# Autodesk Inventor assembly: Robot Réduit
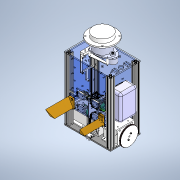
[picture p0: Inventor's stored thumbnail of the model, 180x180]
Saved by Autodesk Inventor 2022 (Build 260153000, 153)
## iProperties
Created: 2022-04-26
Part Number: Robot Réduit
Document SubType Name: Assembly
Designer: victo
Author: victo
## Documents named in this file (25)
- C:\Users\victo\Desktop\Documents\ENSTA\Cours ENSTA\2A\PIE\Modélisation\Robot réduit\Robot Réduit.iam
- C:\Users\victo\Desktop\Documents\ENSTA\Cours ENSTA\2A\PIE\Modélisation\Robot réduit\Base robot réduit.ipt
- C:\Users\victo\Desktop\Documents\ENSTA\Cours ENSTA\2A\PIE\Modélisation\Robot réduit\Biellette moteur-doigts.ipt
- C:\Users\victo\Desktop\Documents\ENSTA\Cours ENSTA\2A\PIE\Modélisation\Robot réduit\Support AX 12A.ipt
- C:\Users\victo\Desktop\Documents\ENSTA\Cours ENSTA\2A\PIE\Modélisation\Propre 0 - Base roue batteries\Moteur déplacement gauche.iam
- C:\Users\victo\Desktop\Documents\ENSTA\Cours ENSTA\2A\PIE\Modélisation\Propre 0 - Base roue batteries\Moteur déplacement droit.iam
- C:\Users\victo\Desktop\Documents\ENSTA\Cours ENSTA\2A\PIE\Modélisation\Robot réduit\Support AX 12A haut.ipt
- C:\Users\victo\Desktop\Documents\ENSTA\Cours ENSTA\2A\PIE\Modélisation\Robot réduit\Batterie et Support Vertical Réduit.iam
- C:\Users\victo\Desktop\Documents\ENSTA\Cours ENSTA\2A\PIE\Modélisation\Robot réduit\Profilés du réduit 20x20.ipt
- C:\Users\victo\Desktop\Documents\ENSTA\Cours ENSTA\2A\PIE\Modélisation\Robot réduit\Support rotation.ipt
- C:\Users\victo\Desktop\Documents\ENSTA\Cours ENSTA\2A\PIE\Modélisation\Robot réduit\Plaque trans.ipt
- C:\Users\victo\Desktop\Documents\ENSTA\Cours ENSTA\2A\PIE\Modélisation\Robot réduit\Doigt droit.ipt
- C:\Users\victo\Desktop\Documents\ENSTA\Cours ENSTA\2A\PIE\Modélisation\Pieces commerce\AX 12AAX-12A_[Servo.ipt
- C:\Users\victo\Desktop\Documents\ENSTA\Cours ENSTA\2A\PIE\Modélisation\Robot réduit\Biellette support-doigts.ipt
- C:\Users\victo\Desktop\Documents\ENSTA\Cours ENSTA\2A\PIE\Modélisation\Robot réduit\Doigt gauche.ipt
- C:\Users\victo\Desktop\Documents\ENSTA\Cours ENSTA\2A\PIE\Modélisation\Robot réduit\Support Vis rotation.ipt
- C:\Users\victo\Desktop\Documents\ENSTA\Cours ENSTA\2A\PIE\Modélisation\Robot réduit\ASS_Roue_Libre-20220506T114758Z-001\ASS_Roue_Libre\ASS_Roue_Libre.iam
- C:\Users\victo\Desktop\Documents\ENSTA\Cours ENSTA\2A\PIE\Modélisation\Robot réduit\Etage robot réduit.ipt
- C:\Users\victo\Desktop\Documents\ENSTA\Cours ENSTA\2A\PIE\Modélisation\Robot réduit\Support_LIDAR.ipt
- C:\Users\victo\Desktop\Documents\ENSTA\Cours ENSTA\2A\PIE\Modélisation\Robot réduit\Support_Raspberry.ipt
- C:\Users\victo\Desktop\Documents\ENSTA\Cours ENSTA\2A\PIE\Modélisation\Robot réduit\Chapeau Haut.stl.ipt
- C:\Users\victo\Desktop\Documents\ENSTA\Cours ENSTA\2A\PIE\Modélisation\Robot réduit\rplidar_main.ipt
- C:\Users\victo\Desktop\Documents\ENSTA\Cours ENSTA\2A\PIE\Modélisation\Robot réduit\Plaques latétales\Plaque avant.ipt
- C:\Users\victo\Desktop\Documents\ENSTA\Cours ENSTA\2A\PIE\Modélisation\Robot réduit\Plaques latétales\Plaque arrière.ipt
- C:\Users\victo\Desktop\Documents\ENSTA\Cours ENSTA\2A\PIE\Modélisation\Robot réduit\Plaques latétales\Plaque gauche.ipt
## Components (35 placed, 24 different names)
1. Base robot réduit:1 — Logement:3, Placage:2, Logement:4, Placage:3, Logement:6, Placage:5, Logement:9, Logement:10, Logement:11, Logement:12, Angle:1, Angle:2, Angle:3, Angle:4, Placage:24, Affleurement:1, Placage:25, Affleurement:2
2. Moteur déplacement droit:1 [sub-assembly] — Logement:4, Placage:3
3. Moteur déplacement gauche:1 [sub-assembly] — Logement:3, Placage:2, Logement:7, Placage:6
4. Support AX 12A:1 — Logement:2, Logement:5, Placage:4, Logement:19, Placage:14, Placage:15, Logement:24, Placage:22
5. Support AX 12A haut:1 — Logement:5, Placage:4, Logement:6, Placage:5, Logement:8, Logement:20, Placage:13, Placage:16, Placage:23, Logement:25
6. Biellette moteur-doigts:1 — Logement:2, Logement:17, Placage:19, Placage:20
7. Batterie et Support Vertical Réduit:1 [sub-assembly] — Logement:7, Placage:6
8. Biellette moteur-doigts:2 — Logement:8, Placage:11, Placage:17, Placage:18
9. Profilés du réduit 20x20:1 — Logement:12, Angle:4
10. Profilés du réduit 20x20:2 — Logement:9, Angle:1, Logement:26
11. Profilés du réduit 20x20:3 — Logement:10, Angle:3, Placage:26
12. Profilés du réduit 20x20:4 — Logement:11, Angle:2
13. Support rotation:1 — Logement:14, Placage:9, Logement:17
14. Support rotation:2 — Logement:13, Placage:10, Logement:22
15. Plaque trans:1 — Logement:13, Logement:14, Logement:15, Logement:16, Placage:7, Placage:8, Placage:9, Placage:10, Logement:18, Placage:12, Logement:23, Placage:21
16. Support rotation:3 — Logement:15, Placage:8, Logement:21
17. Support rotation:4 — Logement:16, Placage:7, Placage:11
18. Doigt droit:1 — Logement:18, Placage:12
19. AX 12AAX-12A_[Servo:1 — Logement:19, Placage:14, Placage:19, Placage:20
20. AX 12AAX-12A_[Servo:2 — Logement:20, Placage:13, Placage:17, Placage:18
21. Biellette support-doigts:1 — Logement:21, Placage:15
22. Biellette support-doigts:2 — Logement:22, Placage:16
23. Doigt gauche:1 — Logement:23, Placage:21
24. Support Vis rotation:1 — Logement:24, Placage:22
25. Support Vis rotation:2 — Placage:23, Logement:25
26. ASS_Roue_Libre:1 [sub-assembly] — Placage:24, Affleurement:1
27. ASS_Roue_Libre:2 [sub-assembly] — Placage:25, Affleurement:2
28. Etage robot réduit:1 — Logement:26, Placage:26, Placage:27, Placage:28, Placage:29, Logement:27, Placage:30, Placage:31, Placage:32, Placage:33, Placage:35, Affleurement:3, Placage:36, Affleurement:38, Placage:37, Affleurement:39
29. Support_LIDAR:1 — Placage:27, Placage:28, Placage:29, Logement:28, Placage:34
30. Support_Raspberry:1 — Logement:27, Placage:30
31. Chapeau Haut.stl:1 — Placage:31, Placage:32, Placage:33
32. rplidar_main:1 — Logement:28, Placage:34
33. Plaque avant:1 — Placage:35, Affleurement:3
34. Plaque arrière:1 — Placage:36, Affleurement:38
35. Plaque gauche:1 — Placage:37, Affleurement:39
## Relationships (72: Mate 36, Insert 27, Flush 5, Angle 4)
- Logement:2 [Insert]: Support AX 12A:1 ↔ Biellette moteur-doigts:1
- Logement:3 [Insert]: Base robot réduit:1 ↔ Moteur déplacement gauche:1
- Placage:2 [Mate]: Base robot réduit:1 ↔ Moteur déplacement gauche:1
- Logement:4 [Insert]: Base robot réduit:1 ↔ Moteur déplacement droit:1
- Placage:3 [Mate]: Base robot réduit:1 ↔ Moteur déplacement droit:1
- Logement:5 [Insert]: Support AX 12A:1 ↔ Support AX 12A haut:1
- Placage:4 [Mate]: Support AX 12A:1 ↔ Support AX 12A haut:1
- Logement:6 [Insert]: Base robot réduit:1 ↔ Support AX 12A haut:1
- Placage:5 [Mate]: Base robot réduit:1 ↔ Support AX 12A haut:1
- Logement:7 [Insert]: Moteur déplacement gauche:1 ↔ Batterie et Support Vertical Réduit:1
- Placage:6 [Mate]: Moteur déplacement gauche:1 ↔ Batterie et Support Vertical Réduit:1
- Logement:8 [Insert]: Support AX 12A haut:1 ↔ Biellette moteur-doigts:2
- Logement:9 [Insert]: Base robot réduit:1 ↔ Profilés du réduit 20x20:2
- Logement:10 [Insert]: Base robot réduit:1 ↔ Profilés du réduit 20x20:3
- Logement:11 [Insert]: Base robot réduit:1 ↔ Profilés du réduit 20x20:4
- Logement:12 [Insert]: Base robot réduit:1 ↔ Profilés du réduit 20x20:1
- Angle:1 (0 deg): Base robot réduit:1 ↔ Profilés du réduit 20x20:2
- Angle:2 (0 deg): Base robot réduit:1 ↔ Profilés du réduit 20x20:4
- Angle:3 (0 deg): Base robot réduit:1 ↔ Profilés du réduit 20x20:3
- Angle:4 (0 deg): Base robot réduit:1 ↔ Profilés du réduit 20x20:1
- Logement:13 [Insert]: Support rotation:2 ↔ Plaque trans:1
- Logement:14 [Insert]: Support rotation:1 ↔ Plaque trans:1
- Logement:15 [Insert]: Plaque trans:1 ↔ Support rotation:3
- Logement:16 [Insert]: Plaque trans:1 ↔ Support rotation:4
- Placage:7 [Mate]: Plaque trans:1 ↔ Support rotation:4
- Placage:8 [Mate]: Plaque trans:1 ↔ Support rotation:3
- Placage:9 [Mate]: Support rotation:1 ↔ Plaque trans:1
- Placage:10 [Mate]: Support rotation:2 ↔ Plaque trans:1
- Logement:17 [Insert] (0.5 mm): Biellette moteur-doigts:1 ↔ Support rotation:1
- Placage:11 [Mate]: Biellette moteur-doigts:2 ↔ Support rotation:4
- Logement:18 [Insert]: Plaque trans:1 ↔ Doigt droit:1
- Placage:12 [Mate]: Plaque trans:1 ↔ Doigt droit:1
- Logement:19 [Insert]: Support AX 12A:1 ↔ AX 12AAX-12A_[Servo:1
- Logement:20 [Insert]: Support AX 12A haut:1 ↔ AX 12AAX-12A_[Servo:2
- Placage:13 [Mate]: Support AX 12A haut:1 ↔ AX 12AAX-12A_[Servo:2
- Placage:14 [Mate]: Support AX 12A:1 ↔ AX 12AAX-12A_[Servo:1
- Logement:21 [Insert] (0.5 mm): Support rotation:3 ↔ Biellette support-doigts:1
- Logement:22 [Insert] (0.5 mm): Support rotation:2 ↔ Biellette support-doigts:2
- Placage:15 [Mate]: Support AX 12A:1 ↔ Biellette support-doigts:1
- Placage:16 [Mate]: Support AX 12A haut:1 ↔ Biellette support-doigts:2
- Placage:17 [Mate]: Biellette moteur-doigts:2 ↔ AX 12AAX-12A_[Servo:2
- Placage:18 [Mate]: Biellette moteur-doigts:2 ↔ AX 12AAX-12A_[Servo:2
- Placage:19 [Mate]: Biellette moteur-doigts:1 ↔ AX 12AAX-12A_[Servo:1
- Placage:20 [Mate]: Biellette moteur-doigts:1 ↔ AX 12AAX-12A_[Servo:1
- Logement:23 [Insert]: Plaque trans:1 ↔ Doigt gauche:1
- Placage:21 [Mate]: Plaque trans:1 ↔ Doigt gauche:1
- Logement:24 [Insert]: Support AX 12A:1 ↔ Support Vis rotation:1
- Placage:22 [Mate]: Support AX 12A:1 ↔ Support Vis rotation:1
- Placage:23 [Mate]: Support AX 12A haut:1 ↔ Support Vis rotation:2
- Logement:25 [Insert]: Support AX 12A haut:1 ↔ Support Vis rotation:2
- Placage:24 [Mate]: Base robot réduit:1 ↔ ASS_Roue_Libre:1
- Affleurement:1 [Flush]: Base robot réduit:1 ↔ ASS_Roue_Libre:1
- Placage:25 [Mate]: Base robot réduit:1 ↔ ASS_Roue_Libre:2
- Affleurement:2 [Flush]: Base robot réduit:1 ↔ ASS_Roue_Libre:2
- Logement:26 [Insert]: Profilés du réduit 20x20:2 ↔ Etage robot réduit:1
- Placage:26 [Mate]: Profilés du réduit 20x20:3 ↔ Etage robot réduit:1
- Placage:27 [Mate]: Etage robot réduit:1 ↔ Support_LIDAR:1
- Placage:28 [Mate]: Etage robot réduit:1 ↔ Support_LIDAR:1
- Placage:29 [Mate]: Etage robot réduit:1 ↔ Support_LIDAR:1
- Logement:27 [Insert]: Etage robot réduit:1 ↔ Support_Raspberry:1
- Placage:30 [Mate]: Etage robot réduit:1 ↔ Support_Raspberry:1
- Placage:31 [Mate]: Etage robot réduit:1 ↔ Chapeau Haut.stl:1
- Placage:32 [Mate]: Etage robot réduit:1 ↔ Chapeau Haut.stl:1
- Placage:33 [Mate] (70 mm): Etage robot réduit:1 ↔ Chapeau Haut.stl:1
- Logement:28 [Insert]: Support_LIDAR:1 ↔ rplidar_main:1
- Placage:34 [Mate]: Support_LIDAR:1 ↔ rplidar_main:1
- Placage:35 [Mate]: Etage robot réduit:1 ↔ Plaque avant:1
- Affleurement:3 [Flush]: Etage robot réduit:1 ↔ Plaque avant:1
- Placage:36 [Mate]: Etage robot réduit:1 ↔ Plaque arrière:1
- Affleurement:38 [Flush]: Etage robot réduit:1 ↔ Plaque arrière:1
- Placage:37 [Mate]: Etage robot réduit:1 ↔ Plaque gauche:1
- Affleurement:39 [Flush]: Etage robot réduit:1 ↔ Plaque gauche:1
